# Autodesk Inventor assembly: S2_Xaxis_500
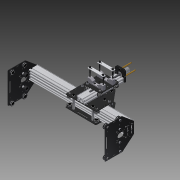
[picture p0: Inventor's stored thumbnail of the model, 180x180]
Saved by Autodesk Inventor 2014 (Build 180170000, 170)
## iProperties
Created: 2013-09-18
Part Number: S2_Xaxis_500
Document SubType Name: Assembly
Designer: Edward
Author: Edward
## Documents named in this file (3)
- C:\Users\Edward\Documents\Vault\Designs\Shapeoko_v2\v2_final\assemblies\S2_Xaxis_500.iam
- C:\Users\Edward\Documents\Vault\Designs\Shapeoko_v2\v2_final\assemblies\S2_Gantry_500.iam
- C:\Users\Edward\Documents\Vault\Designs\Shapeoko_v2\v2_final\assemblies\S2_Zaxis_500.iam
## Components (2 placed, 2 different names)
1. S2_Gantry_500:1 [sub-assembly] — Mate:1, Flush:1
2. S2_Zaxis_500:1 [sub-assembly] — Mate:1, Flush:1
## Relationships (2: Mate 1, Flush 1)
- Mate:1 (6.35 mm): S2_Gantry_500:1 ↔ S2_Zaxis_500:1
- Flush:1 (-25 mm): S2_Gantry_500:1 ↔ S2_Zaxis_500:1
